# Autodesk Inventor assembly: GE-13045R
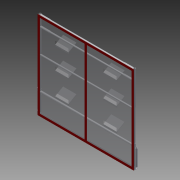
[picture p0: Inventor's stored thumbnail of the model, 180x180]
Saved by Autodesk Inventor 2013 (Build 170138000, 138)
## iProperties
Created: 2013-01-04
Part Number: GE-13045R
Document SubType Name: Assembly
Designer: Phillip
Author: Phillip
## Documents named in this file (9)
- E:\Data Folder\FIRST 2013\FIRST KOP\Field\Feeder Goal Station\GE-13045R.iam
- E:\Data Folder\FIRST 2013\FIRST KOP\Field\Feeder Goal Station\GE-13010.ipt
- E:\Data Folder\FIRST 2013\FIRST KOP\Field\Feeder Goal Station\GE-13015.iam
- E:\Data Folder\FIRST 2013\FIRST KOP\Field\Feeder Goal Station\GE-13035.ipt
- E:\Data Folder\FIRST 2013\FIRST KOP\Field\Feeder Goal Station\GE-13033.iam
- E:\Data Folder\FIRST 2013\FIRST KOP\Field\Feeder Goal Station\GE-13034.ipt
- E:\Data Folder\FIRST 2013\FIRST KOP\Field\Feeder Goal Station\GE-13014.iam
- E:\Data Folder\FIRST 2013\FIRST KOP\Field\Feeder Goal Station\Tape.ipt
- E:\Data Folder\FIRST 2013\FIRST KOP\Field\Feeder Goal Station\GE-13044.ipt
## Components (16 placed, 8 different names)
1. GE-13010:1 — Flush:1, Flush:2, Mate:1, Mate:6, Flush:3, Flush:4, Flush:5, Flush:6, Mate:16, Mate:17, Mate:18, Mate:19, Mate:20, Mate:21, Mate:22, Mate:23, Mate:24
2. GE-13010:2 — Flush:1, Flush:2, Mate:1, Mate:4, Flush:7, Angle:1, Flush:8, Mate:26, Mate:27, Mate:28, Mate:29, Mate:30, Mate:31, Mate:32, Mate:33
3. GE-13015:1 [sub-assembly] — Mate:4, Mate:7, Mate:8, Mate:9, Mate:10
4. GE-13035:1 — Mate:6, Flush:3, Flush:4, Flush:5, Mate:7, Mate:9, Flush:10, Mate:25
5. GE-13033:1 [sub-assembly] — Mate:8, Flush:6, Mate:11, Mate:14
6. GE-13033:2 [sub-assembly] — Mate:10, Flush:7, Angle:1, Mate:11, Mate:12, Mate:13, Mate:15
7. GE-13034:1 — Mate:12
8. GE-13034:2 — Mate:13
9. GE-13014:1 [sub-assembly] — Mate:14, Mate:15
10. Tape:1 — Flush:8, Flush:10
11. GE-13044:1 — Mate:16, Mate:17, Mate:18
12. GE-13044:2 — Mate:19, Mate:20, Mate:21
13. GE-13044:3 — Mate:22, Mate:23, Mate:24
14. GE-13044:4 — Mate:25, Mate:26, Mate:27
15. GE-13044:5 — Mate:28, Mate:29, Mate:30
16. GE-13044:6 — Mate:31, Mate:32, Mate:33
## Relationships (40: Mate 30, Flush 9, Angle 1)
- Flush:1: GE-13010:1 ↔ GE-13010:2
- Flush:2: GE-13010:1 ↔ GE-13010:2
- Mate:1: GE-13010:1 ↔ GE-13010:2
- Mate:4: GE-13010:2 ↔ GE-13015:1
- Mate:6: GE-13010:1 ↔ GE-13035:1
- Flush:3: GE-13010:1 ↔ GE-13035:1
- Flush:4: GE-13010:1 ↔ GE-13035:1
- Flush:5: GE-13010:1 ↔ GE-13035:1
- Mate:7: GE-13015:1 ↔ GE-13035:1
- Mate:8: GE-13015:1 ↔ GE-13033:1
- Flush:6: GE-13010:1 ↔ GE-13033:1
- Mate:9: GE-13015:1 ↔ GE-13035:1
- Mate:10: GE-13015:1 ↔ GE-13033:2
- Flush:7: GE-13010:2 ↔ GE-13033:2
- Angle:1 (0 deg): GE-13010:2 ↔ GE-13033:2
- Mate:11: GE-13033:1 ↔ GE-13033:2
- Mate:12: GE-13033:2 ↔ GE-13034:1
- Mate:13: GE-13033:2 ↔ GE-13034:2
- Mate:14: GE-13033:1 ↔ GE-13014:1
- Mate:15: GE-13033:2 ↔ GE-13014:1
- Flush:8: GE-13010:2 ↔ Tape:1
- Flush:10: GE-13035:1 ↔ Tape:1
- Mate:16: GE-13010:1 ↔ GE-13044:1
- Mate:17: GE-13010:1 ↔ GE-13044:1
- Mate:18 (-38.1 mm): GE-13010:1 ↔ GE-13044:1
- Mate:19: GE-13010:1 ↔ GE-13044:2
- Mate:20: GE-13010:1 ↔ GE-13044:2
- Mate:21 (-38.1 mm): GE-13010:1 ↔ GE-13044:2
- Mate:22: GE-13010:1 ↔ GE-13044:3
- Mate:23: GE-13010:1 ↔ GE-13044:3
- Mate:24 (-38.1 mm): GE-13010:1 ↔ GE-13044:3
- Mate:25: GE-13035:1 ↔ GE-13044:4
- Mate:26: GE-13010:2 ↔ GE-13044:4
- Mate:27 (-38.1 mm): GE-13010:2 ↔ GE-13044:4
- Mate:28: GE-13010:2 ↔ GE-13044:5
- Mate:29: GE-13010:2 ↔ GE-13044:5
- Mate:30 (-38.1 mm): GE-13010:2 ↔ GE-13044:5
- Mate:31: GE-13010:2 ↔ GE-13044:6
- Mate:32: GE-13010:2 ↔ GE-13044:6
- Mate:33 (-38.1 mm): GE-13010:2 ↔ GE-13044:6
